# Autodesk Inventor assembly: Assembly1
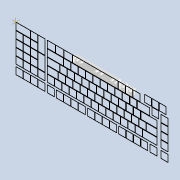
[picture p0: Inventor's stored thumbnail of the model, 180x180]
Saved by Autodesk Inventor 2021 (Build 250183000, 183)
## iProperties
Created: 2021-12-04
Part Number: Assembly1
Document SubType Name: Assembly
Designer: Matthew Flooks
Author: Matthew Flooks
## Documents named in this file (5)
- C:\Users\Matthew Flooks\Documents\GitHub\QEX103-PCB\3D Model\Assembly1.iam
- C:\Users\Matthew Flooks\Documents\GitHub\QEX103-PCB\3D Model\Layout.ipt
- C:\Users\Matthew Flooks\Documents\GitHub\QEX103-PCB\3D Model\KeyCaps\Space.ipt
- C:\Users\Matthew Flooks\Documents\GitHub\QEX103-PCB\3D Model\KeyCaps\AltLeft.ipt
- C:\Users\Matthew Flooks\Documents\GitHub\QEX103-PCB\3D Model\KeyCaps\CtrlLeft.ipt
## Components (4 placed, 4 different names)
1. Layout:1 — Mate:1, Mate:2, Mate:3, Mate:4, Mate:5, Mate:6, Mate:7, Mate:8
2. Space:1 — Mate:3, Mate:4
3. AltLeft:1 — Mate:5, Mate:6
4. CtrlLeft:1 — Mate:7, Mate:8
## Relationships (8: Mate 8)
- Mate:1: Layout:1
- Mate:2: Layout:1
- Mate:3: Layout:1 ↔ Space:1
- Mate:4: Layout:1 ↔ Space:1
- Mate:5: Layout:1 ↔ AltLeft:1
- Mate:6: Layout:1 ↔ AltLeft:1
- Mate:7: Layout:1 ↔ CtrlLeft:1
- Mate:8: Layout:1 ↔ CtrlLeft:1
